# Autodesk Inventor assembly: rover assembly
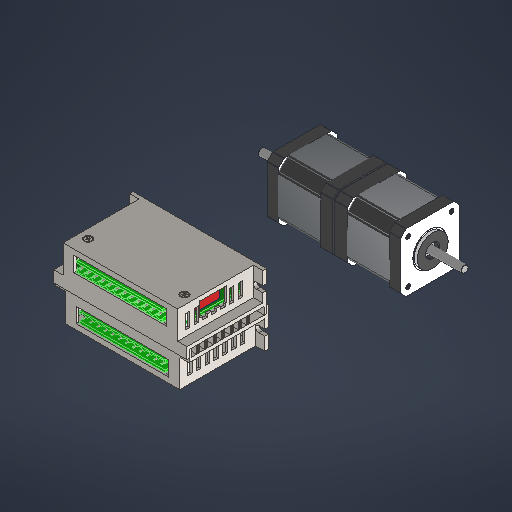
[picture p0: Inventor's stored thumbnail of the model, 512x512]
Saved by Autodesk Inventor 2026.3 (Build 303398000, 398)
## iProperties
Created: 2026-04-19
Part Number: rover assembly
Document SubType Name: Assembly
Designer: micha
Author: micha
## Documents named in this file (3)
- C:\Users\micha\Documents\Inventor\Robot-Mower\rover assembly.iam
- C:\Users\micha\Documents\Inventor\Robot-Mower\tb6600-stepper-motor-driver-3.snapshot.5\Assembly\Assembly.iam
- C:\Users\micha\Documents\Inventor\Robot-Mower\nema17-4-4kgcm-stepper-motor-1.snapshot.1\Nema17 4.4Kgcm Stepper Motor\Nema17 4.4Kgcm Stepper Motor.iam
## Components (4 placed, 2 different names)
1. Assembly:1 [sub-assembly] — Mate:1, Mate:2, Mate:3, Flush:1, Flush:3
2. Assembly:2 [sub-assembly] — Mate:1, Mate:2, Mate:4, Flush:1, Flush:2
3. Nema17 4.4Kgcm Stepper Motor:1 [sub-assembly] — Flush:2, Flush:4, Flush:5
4. Nema17 4.4Kgcm Stepper Motor:2 [sub-assembly] — Flush:3, Flush:4, Flush:5
## Relationships (9: Flush 5, Mate 4)
- Mate:1: Assembly:1 ↔ Assembly:2
- Mate:2: Assembly:1 ↔ Assembly:2
- Mate:3: Assembly:1
- Mate:4: Assembly:2
- Flush:1: Assembly:1 ↔ Assembly:2
- Flush:2: Assembly:2 ↔ Nema17 4.4Kgcm Stepper Motor:1
- Flush:3: Assembly:1 ↔ Nema17 4.4Kgcm Stepper Motor:2
- Flush:4: Nema17 4.4Kgcm Stepper Motor:1 ↔ Nema17 4.4Kgcm Stepper Motor:2
- Flush:5: Nema17 4.4Kgcm Stepper Motor:1 ↔ Nema17 4.4Kgcm Stepper Motor:2
